# Autodesk Inventor assembly: Assembly1
(part 3 of 8)
- [Mate]: disk holder:43 ↔ Coil:85
- [Mate]: disk holder:43 ↔ Coil:85
- [Angle] (270 deg): disk holder:43 ↔ Coil:85
- [Mate]: disk holder:43 ↔ Coil:86
- [Angle] (270 deg): disk holder:43 ↔ Coil:86
- [Mate]: disk holder:43 ↔ Coil:86
- [RevoluteJoint]: disk holder:44 ↔ coin:44
- [Angle] (-25 deg): disk holder:44 ↔ coin:44
- [Mate]: disk holder:44 ↔ Coil:87
- [Mate]: disk holder:44 ↔ Coil:87
- [Angle] (270 deg): disk holder:44 ↔ Coil:87
- [Mate]: disk holder:44 ↔ Coil:88
- [Angle] (270 deg): disk holder:44 ↔ Coil:88
- [Mate]: disk holder:44 ↔ Coil:88
- [RevoluteJoint]: disk holder:45 ↔ coin:45
- [Angle] (-25 deg): disk holder:45 ↔ coin:45
- [Mate]: disk holder:45 ↔ Coil:89
- [Mate]: disk holder:45 ↔ Coil:89
- [Angle] (270 deg): disk holder:45 ↔ Coil:89
- [Mate]: disk holder:45 ↔ Coil:90
- [Angle] (270 deg): disk holder:45 ↔ Coil:90
- [Mate]: disk holder:45 ↔ Coil:90
- Flush:37: FRAME:1 ↔ disk holder:42
- Flush:38: FRAME:1 ↔ disk holder:43
- Flush:39: FRAME:1 ↔ disk holder:41
- Flush:40: FRAME:1 ↔ disk holder:38
- Mate:271: FRAME:1 ↔ disk holder:38
- Mate:272: FRAME:1 ↔ disk holder:38
- Flush:41: FRAME:1 ↔ disk holder:39
- Flush:42: FRAME:1 ↔ disk holder:45
- Flush:43: FRAME:1 ↔ disk holder:44
- Mate:277: FRAME:1 ↔ disk holder:44
- Mate:278: FRAME:1 ↔ disk holder:44
- Flush:44: FRAME:1 ↔ disk holder:40
- [RevoluteJoint]: disk holder:46 ↔ coin:46
- [Angle] (-25 deg): disk holder:46 ↔ coin:46
- [Mate]: disk holder:46 ↔ Coil:91
- [Mate]: disk holder:46 ↔ Coil:91
- [Angle] (270 deg): disk holder:46 ↔ Coil:91
- [Mate]: disk holder:46 ↔ Coil:92
- [Angle] (270 deg): disk holder:46 ↔ Coil:92
- [Mate]: disk holder:46 ↔ Coil:92
- [RevoluteJoint]: disk holder:47 ↔ coin:47
- [Angle] (-25 deg): disk holder:47 ↔ coin:47
- [Mate]: disk holder:47 ↔ Coil:93
- [Mate]: disk holder:47 ↔ Coil:93
- [Angle] (270 deg): disk holder:47 ↔ Coil:93
- [Mate]: disk holder:47 ↔ Coil:94
- [Angle] (270 deg): disk holder:47 ↔ Coil:94
- [Mate]: disk holder:47 ↔ Coil:94
- [RevoluteJoint]: disk holder:48 ↔ coin:48
- [Angle] (-25 deg): disk holder:48 ↔ coin:48
- [Mate]: disk holder:48 ↔ Coil:95
- [Mate]: disk holder:48 ↔ Coil:95
- [Angle] (270 deg): disk holder:48 ↔ Coil:95
- [Mate]: disk holder:48 ↔ Coil:96
- [Angle] (270 deg): disk holder:48 ↔ Coil:96
- [Mate]: disk holder:48 ↔ Coil:96
- [RevoluteJoint]: disk holder:50 ↔ coin:50
- [Angle] (-25 deg): disk holder:50 ↔ coin:50
- [Mate]: disk holder:50 ↔ Coil:99
- [Mate]: disk holder:50 ↔ Coil:99
- [Angle] (270 deg): disk holder:50 ↔ Coil:99
- [Mate]: disk holder:50 ↔ Coil:100
- [Angle] (270 deg): disk holder:50 ↔ Coil:100
- [Mate]: disk holder:50 ↔ Coil:100
- [RevoluteJoint]: disk holder:51 ↔ coin:51
- [Angle] (-25 deg): disk holder:51 ↔ coin:51
- [Mate]: disk holder:51 ↔ Coil:101
- [Mate]: disk holder:51 ↔ Coil:101
- [Angle] (270 deg): disk holder:51 ↔ Coil:101
- [Mate]: disk holder:51 ↔ Coil:102
- [Angle] (270 deg): disk holder:51 ↔ Coil:102
- [Mate]: disk holder:51 ↔ Coil:102
- [RevoluteJoint]: disk holder:53 ↔ coin:53
- [Angle] (-25 deg): disk holder:53 ↔ coin:53
- [Mate]: disk holder:53 ↔ Coil:105
- [Mate]: disk holder:53 ↔ Coil:105
- [Angle] (270 deg): disk holder:53 ↔ Coil:105
- [Mate]: disk holder:53 ↔ Coil:106
- [Angle] (270 deg): disk holder:53 ↔ Coil:106
- [Mate]: disk holder:53 ↔ Coil:106
- [RevoluteJoint]: disk holder:55 ↔ coin:55
- [Angle] (-25 deg): disk holder:55 ↔ coin:55
- [Mate]: disk holder:55 ↔ Coil:109
- [Mate]: disk holder:55 ↔ Coil:109
- [Angle] (270 deg): disk holder:55 ↔ Coil:109
- [Mate]: disk holder:55 ↔ Coil:110
- [Angle] (270 deg): disk holder:55 ↔ Coil:110
- [Mate]: disk holder:55 ↔ Coil:110
- [RevoluteJoint]: disk holder:57 ↔ coin:57
- [Angle] (-25 deg): disk holder:57 ↔ coin:57
- [Mate]: disk holder:57 ↔ Coil:113
- [Mate]: disk holder:57 ↔ Coil:113
- [Angle] (270 deg): disk holder:57 ↔ Coil:113
- [Mate]: disk holder:57 ↔ Coil:114
- [Angle] (270 deg): disk holder:57 ↔ Coil:114
- [Mate]: disk holder:57 ↔ Coil:114
- Flush:45: disk holder:46 ↔ disk holder:48
- Flush:46: disk holder:47 ↔ disk holder:48
- Flush:49: disk holder:50 ↔ disk holder:51
- Flush:59: disk holder:55 ↔ disk holder:57
- Flush:60: disk holder:53 ↔ disk holder:57
- Flush:61: disk holder:51 ↔ disk holder:55
- Flush:62: disk holder:50 ↔ disk holder:55
- Mate:335: FRAME:1 ↔ disk holder:48
- Mate:338: FRAME:1 ↔ disk holder:47
- Mate:339: FRAME:1 ↔ disk holder:55
- Mate:340: FRAME:1 ↔ disk holder:51
- Mate:343: FRAME:1 ↔ disk holder:53
- Mate:344: FRAME:1 ↔ disk holder:57
- Mate:345: FRAME:1 ↔ disk holder:50
- [RevoluteJoint]: disk holder:59 ↔ coin:59
- [Angle] (-25 deg): disk holder:59 ↔ coin:59
- [Mate]: disk holder:59 ↔ Coil:117
- [Mate]: disk holder:59 ↔ Coil:117
- [Angle] (270 deg): disk holder:59 ↔ Coil:117
- [Mate]: disk holder:59 ↔ Coil:118
- [Angle] (270 deg): disk holder:59 ↔ Coil:118
- [Mate]: disk holder:59 ↔ Coil:118
- [RevoluteJoint]: disk holder:60 ↔ coin:60
- [Angle] (-25 deg): disk holder:60 ↔ coin:60
- [Mate]: disk holder:60 ↔ Coil:119
- [Mate]: disk holder:60 ↔ Coil:119
- [Angle] (270 deg): disk holder:60 ↔ Coil:119
- [Mate]: disk holder:60 ↔ Coil:120
- [Angle] (270 deg): disk holder:60 ↔ Coil:120
- [Mate]: disk holder:60 ↔ Coil:120
- [RevoluteJoint]: disk holder:61 ↔ coin:61
- [Angle] (-25 deg): disk holder:61 ↔ coin:61
- [Mate]: disk holder:61 ↔ Coil:121
- [Mate]: disk holder:61 ↔ Coil:121
- [Angle] (270 deg): disk holder:61 ↔ Coil:121
- [Mate]: disk holder:61 ↔ Coil:122
- [Angle] (270 deg): disk holder:61 ↔ Coil:122
- [Mate]: disk holder:61 ↔ Coil:122
- [RevoluteJoint]: disk holder:62 ↔ coin:62
- [Angle] (-25 deg): disk holder:62 ↔ coin:62
- [Mate]: disk holder:62 ↔ Coil:123
- [Mate]: disk holder:62 ↔ Coil:123
- [Angle] (270 deg): disk holder:62 ↔ Coil:123
- [Mate]: disk holder:62 ↔ Coil:124
- [Angle] (270 deg): disk holder:62 ↔ Coil:124
- [Mate]: disk holder:62 ↔ Coil:124
- [RevoluteJoint]: disk holder:63 ↔ coin:63
- [Angle] (-25 deg): disk holder:63 ↔ coin:63
- [Mate]: disk holder:63 ↔ Coil:125
- [Mate]: disk holder:63 ↔ Coil:125
- [Angle] (270 deg): disk holder:63 ↔ Coil:125
- [Mate]: disk holder:63 ↔ Coil:126
- [Angle] (270 deg): disk holder:63 ↔ Coil:126
- [Mate]: disk holder:63 ↔ Coil:126
- [RevoluteJoint]: disk holder:64 ↔ coin:64
- [Angle] (-25 deg): disk holder:64 ↔ coin:64
- [Mate]: disk holder:64 ↔ Coil:127
- [Mate]: disk holder:64 ↔ Coil:127
- [Angle] (270 deg): disk holder:64 ↔ Coil:127
- [Mate]: disk holder:64 ↔ Coil:128
- [Angle] (270 deg): disk holder:64 ↔ Coil:128
- [Mate]: disk holder:64 ↔ Coil:128
- [RevoluteJoint]: disk holder:65 ↔ coin:65
- [Angle] (-25 deg): disk holder:65 ↔ coin:65
- [Mate]: disk holder:65 ↔ Coil:129
- [Mate]: disk holder:65 ↔ Coil:129
- [Angle] (270 deg): disk holder:65 ↔ Coil:129
- [Mate]: disk holder:65 ↔ Coil:130
- [Angle] (270 deg): disk holder:65 ↔ Coil:130
- [Mate]: disk holder:65 ↔ Coil:130
- [RevoluteJoint]: disk holder:66 ↔ coin:66
- [Angle] (-25 deg): disk holder:66 ↔ coin:66
- [Mate]: disk holder:66 ↔ Coil:131
- [Mate]: disk holder:66 ↔ Coil:131
- [Angle] (270 deg): disk holder:66 ↔ Coil:131
- [Mate]: disk holder:66 ↔ Coil:132
- [Angle] (270 deg): disk holder:66 ↔ Coil:132
- [Mate]: disk holder:66 ↔ Coil:132
- [RevoluteJoint]: disk holder:67 ↔ coin:67
- [Angle] (-25 deg): disk holder:67 ↔ coin:67
- [Mate]: disk holder:67 ↔ Coil:133
- [Mate]: disk holder:67 ↔ Coil:133
- [Angle] (270 deg): disk holder:67 ↔ Coil:133
- [Mate]: disk holder:67 ↔ Coil:134
- [Angle] (270 deg): disk holder:67 ↔ Coil:134
- [Mate]: disk holder:67 ↔ Coil:134
- [RevoluteJoint]: disk holder:68 ↔ coin:68
- [Angle] (-25 deg): disk holder:68 ↔ coin:68
- [Mate]: disk holder:68 ↔ Coil:135
- [Mate]: disk holder:68 ↔ Coil:135
- [Angle] (270 deg): disk holder:68 ↔ Coil:135
- [Mate]: disk holder:68 ↔ Coil:136
- [Angle] (270 deg): disk holder:68 ↔ Coil:136
- [Mate]: disk holder:68 ↔ Coil:136
- [RevoluteJoint]: disk holder:69 ↔ coin:69
- [Angle] (-25 deg): disk holder:69 ↔ coin:69
- [Mate]: disk holder:69 ↔ Coil:137
- [Mate]: disk holder:69 ↔ Coil:137
- [Angle] (270 deg): disk holder:69 ↔ Coil:137
- [Mate]: disk holder:69 ↔ Coil:138
- [Angle] (270 deg): disk holder:69 ↔ Coil:138
- [Mate]: disk holder:69 ↔ Coil:138
- Flush:71: disk holder:46 ↔ disk holder:61
- Flush:72: disk holder:61 ↔ disk holder:64
- Flush:73: disk holder:59 ↔ disk holder:64
- Flush:74: disk holder:59 ↔ disk holder:60
- Flush:75: disk holder:60 ↔ disk holder:62
- Flush:76: disk holder:60 ↔ disk holder:68
- Flush:77: disk holder:60 ↔ disk holder:63
- Flush:78: disk holder:63 ↔ disk holder:66
- Flush:79: disk holder:62 ↔ disk holder:65
- Flush:80: disk holder:65 ↔ disk holder:67
- Flush:81: disk holder:67 ↔ disk holder:69
- Flush:82: disk holder:46 ↔ disk holder:61
- Flush:83: disk holder:46 ↔ disk holder:62
- Flush:84: disk holder:46 ↔ disk holder:60
- Flush:85: disk holder:61 ↔ disk holder:65
- Flush:86: disk holder:64 ↔ disk holder:66
- Flush:88: disk holder:63 ↔ disk holder:67
- Flush:89: disk holder:68 ↔ disk holder:69
- Flush:90: disk holder:64 ↔ disk holder:67
- Flush:91: disk holder:64 ↔ disk holder:69
- Flush:92: disk holder:60 ↔ disk holder:67
- Mate:390: FRAME:1 ↔ disk holder:69
- Mate:391: FRAME:1 ↔ disk holder:69
- Mate:392: FRAME:1 ↔ disk holder:68
- Mate:393: FRAME:1 ↔ disk holder:61
- Mate:394: FRAME:1 ↔ disk holder:46
- Mate:395: FRAME:1 ↔ disk holder:60
- Mate:396: FRAME:1 ↔ disk holder:65
- Mate:397: FRAME:1 ↔ disk holder:62
- Mate:398: FRAME:1 ↔ disk holder:67
- Mate:399: FRAME:1 ↔ disk holder:63
- Mate:400: FRAME:1 ↔ disk holder:64
- Mate:401: FRAME:1 ↔ disk holder:66
- [RevoluteJoint]: disk holder:70 ↔ coin:70
- [Angle] (-25 deg): disk holder:70 ↔ coin:70
- [Mate]: disk holder:70 ↔ Coil:139
- [Mate]: disk holder:70 ↔ Coil:139
- [Angle] (270 deg): disk holder:70 ↔ Coil:139
- [Mate]: disk holder:70 ↔ Coil:140
- [Angle] (270 deg): disk holder:70 ↔ Coil:140
- [Mate]: disk holder:70 ↔ Coil:140
- [RevoluteJoint]: disk holder:71 ↔ coin:71
- [Angle] (-25 deg): disk holder:71 ↔ coin:71
- [Mate]: disk holder:71 ↔ Coil:141
- [Mate]: disk holder:71 ↔ Coil:141
- [Angle] (270 deg): disk holder:71 ↔ Coil:141
- [Mate]: disk holder:71 ↔ Coil:142
- [Angle] (270 deg): disk holder:71 ↔ Coil:142
- [Mate]: disk holder:71 ↔ Coil:142
- [RevoluteJoint]: disk holder:72 ↔ coin:72
- [Angle] (-25 deg): disk holder:72 ↔ coin:72
- [Mate]: disk holder:72 ↔ Coil:143
- [Mate]: disk holder:72 ↔ Coil:143
- [Angle] (270 deg): disk holder:72 ↔ Coil:143
- [Mate]: disk holder:72 ↔ Coil:144
- [Angle] (270 deg): disk holder:72 ↔ Coil:144
- [Mate]: disk holder:72 ↔ Coil:144
- [RevoluteJoint]: disk holder:74 ↔ coin:74
- [Angle] (-25 deg): disk holder:74 ↔ coin:74
- [Mate]: disk holder:74 ↔ Coil:147
- [Mate]: disk holder:74 ↔ Coil:147
- [Angle] (270 deg): disk holder:74 ↔ Coil:147
- [Mate]: disk holder:74 ↔ Coil:148
- [Angle] (270 deg): disk holder:74 ↔ Coil:148
- [Mate]: disk holder:74 ↔ Coil:148
- [RevoluteJoint]: disk holder:75 ↔ coin:75
- [Angle] (-25 deg): disk holder:75 ↔ coin:75
- [Mate]: disk holder:75 ↔ Coil:149
- [Mate]: disk holder:75 ↔ Coil:149
- [Angle] (270 deg): disk holder:75 ↔ Coil:149
- [Mate]: disk holder:75 ↔ Coil:150
- [Angle] (270 deg): disk holder:75 ↔ Coil:150
- [Mate]: disk holder:75 ↔ Coil:150
- [RevoluteJoint]: disk holder:76 ↔ coin:76
- [Angle] (-25 deg): disk holder:76 ↔ coin:76
- [Mate]: disk holder:76 ↔ Coil:151
- [Mate]: disk holder:76 ↔ Coil:151
- [Angle] (270 deg): disk holder:76 ↔ Coil:151
- [Mate]: disk holder:76 ↔ Coil:152
- [Angle] (270 deg): disk holder:76 ↔ Coil:152
- [Mate]: disk holder:76 ↔ Coil:152
- [RevoluteJoint]: disk holder:77 ↔ coin:77
- [Angle] (-25 deg): disk holder:77 ↔ coin:77
- [Mate]: disk holder:77 ↔ Coil:153
- [Mate]: disk holder:77 ↔ Coil:153
- [Angle] (270 deg): disk holder:77 ↔ Coil:153
- [Mate]: disk holder:77 ↔ Coil:154
- [Angle] (270 deg): disk holder:77 ↔ Coil:154
- [Mate]: disk holder:77 ↔ Coil:154
- [RevoluteJoint]: disk holder:78 ↔ coin:78
- [Angle] (-25 deg): disk holder:78 ↔ coin:78
- [Mate]: disk holder:78 ↔ Coil:155
- [Mate]: disk holder:78 ↔ Coil:155
- [Angle] (270 deg): disk holder:78 ↔ Coil:155
- [Mate]: disk holder:78 ↔ Coil:156
- [Angle] (270 deg): disk holder:78 ↔ Coil:156
- [Mate]: disk holder:78 ↔ Coil:156
- [RevoluteJoint]: disk holder:79 ↔ coin:79
- [Angle] (-25 deg): disk holder:79 ↔ coin:79
- [Mate]: disk holder:79 ↔ Coil:157
- [Mate]: disk holder:79 ↔ Coil:157
- [Angle] (270 deg): disk holder:79 ↔ Coil:157
- [Mate]: disk holder:79 ↔ Coil:158
- [Angle] (270 deg): disk holder:79 ↔ Coil:158
- [Mate]: disk holder:79 ↔ Coil:158
- [RevoluteJoint]: disk holder:80 ↔ coin:80
- [Angle] (-25 deg): disk holder:80 ↔ coin:80
- [Mate]: disk holder:80 ↔ Coil:159
- [Mate]: disk holder:80 ↔ Coil:159
- [Angle] (270 deg): disk holder:80 ↔ Coil:159
- [Mate]: disk holder:80 ↔ Coil:160
- [Angle] (270 deg): disk holder:80 ↔ Coil:160
- [Mate]: disk holder:80 ↔ Coil:160
- [RevoluteJoint]: disk holder:81 ↔ coin:81
- [Angle] (-25 deg): disk holder:81 ↔ coin:81
- [Mate]: disk holder:81 ↔ Coil:161
- [Mate]: disk holder:81 ↔ Coil:161
- [Angle] (270 deg): disk holder:81 ↔ Coil:161
- [Mate]: disk holder:81 ↔ Coil:162
- [Angle] (270 deg): disk holder:81 ↔ Coil:162
- [Mate]: disk holder:81 ↔ Coil:162
- Flush:94: disk holder:59 ↔ disk holder:74
- Flush:95: disk holder:74 ↔ disk holder:75
- Flush:96: disk holder:72 ↔ disk holder:74
- Flush:97: disk holder:59 ↔ disk holder:70
- Flush:98: disk holder:71 ↔ disk holder:74
- Flush:99: disk holder:72 ↔ disk holder:77
- Flush:100: disk holder:76 ↔ disk holder:77
- Flush:101: disk holder:77 ↔ disk holder:78
- Flush:102: disk holder:76 ↔ disk holder:79
- Flush:103: disk holder:80 ↔ disk holder:81
- Flush:104: disk holder:76 ↔ disk holder:80
- Flush:105: disk holder:78 ↔ disk holder:79
- Flush:106: disk holder:79 ↔ disk holder:81
- Flush:107: disk holder:77 ↔ disk holder:81
- Flush:108: disk holder:77 ↔ disk holder:80
- Flush:109: disk holder:76 ↔ disk holder:80
- Flush:110: disk holder:71 ↔ disk holder:76
- Flush:111: disk holder:71 ↔ disk holder:75
- Flush:112: disk holder:74 ↔ disk holder:75
- Flush:113: disk holder:72 ↔ disk holder:74
- Flush:114: disk holder:59 ↔ disk holder:72
- Mate:450: FRAME:1 ↔ disk holder:70
- Mate:451: FRAME:1 ↔ disk holder:74
- Mate:452: FRAME:1 ↔ disk holder:78
- Mate:453: FRAME:1 ↔ disk holder:77
- Mate:454: FRAME:1 ↔ disk holder:70
- Mate:455: FRAME:1 ↔ disk holder:72
- Mate:456: FRAME:1 ↔ disk holder:80
- Mate:457: FRAME:1 ↔ disk holder:81
- Mate:458: FRAME:1 ↔ disk holder:79
- Mate:459: FRAME:1 ↔ disk holder:75
- Mate:460: FRAME:1 ↔ disk holder:59
- Mate:461: FRAME:1 ↔ disk holder:71
- Mate:462: FRAME:1 ↔ disk holder:76
- [RevoluteJoint]: disk holder:82 ↔ coin:82
- [Angle] (-25 deg): disk holder:82 ↔ coin:82
- [Mate]: disk holder:82 ↔ Coil:163
- [Mate]: disk holder:82 ↔ Coil:163
- [Angle] (270 deg): disk holder:82 ↔ Coil:163
- [Mate]: disk holder:82 ↔ Coil:164
- [Angle] (270 deg): disk holder:82 ↔ Coil:164
- [Mate]: disk holder:82 ↔ Coil:164
- [RevoluteJoint]: disk holder:83 ↔ coin:83
- [Angle] (-25 deg): disk holder:83 ↔ coin:83
- [Mate]: disk holder:83 ↔ Coil:165
- [Mate]: disk holder:83 ↔ Coil:165
- [Angle] (270 deg): disk holder:83 ↔ Coil:165
- [Mate]: disk holder:83 ↔ Coil:166
- [Angle] (270 deg): disk holder:83 ↔ Coil:166
- [Mate]: disk holder:83 ↔ Coil:166
- [RevoluteJoint]: disk holder:84 ↔ coin:84
- [Angle] (-25 deg): disk holder:84 ↔ coin:84
- [Mate]: disk holder:84 ↔ Coil:167
- [Mate]: disk holder:84 ↔ Coil:167
- [Angle] (270 deg): disk holder:84 ↔ Coil:167
- [Mate]: disk holder:84 ↔ Coil:168
- [Angle] (270 deg): disk holder:84 ↔ Coil:168
- [Mate]: disk holder:84 ↔ Coil:168
- [RevoluteJoint]: disk holder:85 ↔ coin:85
- [Angle] (-25 deg): disk holder:85 ↔ coin:85
- [Mate]: disk holder:85 ↔ Coil:169
- [Mate]: disk holder:85 ↔ Coil:169
- [Angle] (270 deg): disk holder:85 ↔ Coil:169
- [Mate]: disk holder:85 ↔ Coil:170
- [Angle] (270 deg): disk holder:85 ↔ Coil:170
- [Mate]: disk holder:85 ↔ Coil:170
- [RevoluteJoint]: disk holder:86 ↔ coin:86
- [Angle] (-25 deg): disk holder:86 ↔ coin:86
- [Mate]: disk holder:86 ↔ Coil:171
- [Mate]: disk holder:86 ↔ Coil:171
- [Angle] (270 deg): disk holder:86 ↔ Coil:171
- [Mate]: disk holder:86 ↔ Coil:172
- [Angle] (270 deg): disk holder:86 ↔ Coil:172
- [Mate]: disk holder:86 ↔ Coil:172
- [RevoluteJoint]: disk holder:87 ↔ coin:87
- [Angle] (-25 deg): disk holder:87 ↔ coin:87
- [Mate]: disk holder:87 ↔ Coil:173
- [Mate]: disk holder:87 ↔ Coil:173
- [Angle] (270 deg): disk holder:87 ↔ Coil:173
- [Mate]: disk holder:87 ↔ Coil:174
- [Angle] (270 deg): disk holder:87 ↔ Coil:174
- [Mate]: disk holder:87 ↔ Coil:174
- [RevoluteJoint]: disk holder:88 ↔ coin:88
- [Angle] (-25 deg): disk holder:88 ↔ coin:88
- [Mate]: disk holder:88 ↔ Coil:175
- [Mate]: disk holder:88 ↔ Coil:175
- [Angle] (270 deg): disk holder:88 ↔ Coil:175
- [Mate]: disk holder:88 ↔ Coil:176
- [Angle] (270 deg): disk holder:88 ↔ Coil:176
- [Mate]: disk holder:88 ↔ Coil:176
- [RevoluteJoint]: disk holder:89 ↔ coin:89
- [Angle] (-25 deg): disk holder:89 ↔ coin:89
- [Mate]: disk holder:89 ↔ Coil:177
- [Mate]: disk holder:89 ↔ Coil:177
- [Angle] (270 deg): disk holder:89 ↔ Coil:177
- [Mate]: disk holder:89 ↔ Coil:178
- [Angle] (270 deg): disk holder:89 ↔ Coil:178
- [Mate]: disk holder:89 ↔ Coil:178
- [RevoluteJoint]: disk holder:90 ↔ coin:90
- [Angle] (-25 deg): disk holder:90 ↔ coin:90
- [Mate]: disk holder:90 ↔ Coil:179
- [Mate]: disk holder:90 ↔ Coil:179
- [Angle] (270 deg): disk holder:90 ↔ Coil:179
- [Mate]: disk holder:90 ↔ Coil:180
- [Angle] (270 deg): disk holder:90 ↔ Coil:180
- [Mate]: disk holder:90 ↔ Coil:180
- Flush:117: FRAME:1 ↔ disk holder:82
- Flush:118: disk holder:82 ↔ disk holder:83
- Flush:119: disk holder:83 ↔ disk holder:84
- Flush:120: disk holder:84 ↔ disk holder:85
- Flush:121: disk holder:85 ↔ disk holder:86
- Flush:122: disk holder:86 ↔ disk holder:87
- Flush:123: disk holder:87 ↔ disk holder:88
- Flush:124: disk holder:88 ↔ disk holder:89
- Flush:125: disk holder:89 ↔ disk holder:90
- Flush:126: disk holder:82 ↔ disk holder:83
- Flush:127: disk holder:83 ↔ disk holder:84
- Flush:128: disk holder:84 ↔ disk holder:85
- Flush:129: disk holder:85 ↔ disk holder:86
- Flush:130: disk holder:86 ↔ disk holder:87
- Flush:131: disk holder:87 ↔ disk holder:88
- Flush:132: disk holder:88 ↔ disk holder:89
- Flush:133: disk holder:89 ↔ disk holder:90
- Mate:499: FRAME:1 ↔ disk holder:82
- Mate:500: FRAME:1 ↔ disk holder:82
- Mate:501: FRAME:1 ↔ disk holder:83
- Mate:502: FRAME:1 ↔ disk holder:84
- Mate:503: FRAME:1 ↔ disk holder:85
- Mate:504: FRAME:1 ↔ disk holder:86
- Mate:505: FRAME:1 ↔ disk holder:87
- Mate:506: FRAME:1 ↔ disk holder:88
- Mate:507: FRAME:1 ↔ disk holder:89
- Mate:508: FRAME:1 ↔ disk holder:90
- [RevoluteJoint]: disk holder:91 ↔ coin:91
- [Angle] (-25 deg): disk holder:91 ↔ coin:91
- [Mate]: disk holder:91 ↔ Coil:181
- [Mate]: disk holder:91 ↔ Coil:181
- [Angle] (270 deg): disk holder:91 ↔ Coil:181
- [Mate]: disk holder:91 ↔ Coil:182
- [Angle] (270 deg): disk holder:91 ↔ Coil:182
- [Mate]: disk holder:91 ↔ Coil:182
- Flush:134: FRAME:1 ↔ disk holder:91
- Mate:513: FRAME:1 ↔ disk holder:91
- Mate:514: FRAME:1 ↔ disk holder:91
- [RevoluteJoint]: disk holder:92 ↔ coin:92
- [Angle] (-25 deg): disk holder:92 ↔ coin:92
- [Mate]: disk holder:92 ↔ Coil:183
- [Mate]: disk holder:92 ↔ Coil:183
- [Angle] (270 deg): disk holder:92 ↔ Coil:183
- [Mate]: disk holder:92 ↔ Coil:184
- [Angle] (270 deg): disk holder:92 ↔ Coil:184
- [Mate]: disk holder:92 ↔ Coil:184
- [RevoluteJoint]: disk holder:93 ↔ coin:93
- [Angle] (-25 deg): disk holder:93 ↔ coin:93
- [Mate]: disk holder:93 ↔ Coil:185
- [Mate]: disk holder:93 ↔ Coil:185
- [Angle] (270 deg): disk holder:93 ↔ Coil:185
- [Mate]: disk holder:93 ↔ Coil:186
- [Angle] (270 deg): disk holder:93 ↔ Coil:186
- [Mate]: disk holder:93 ↔ Coil:186
- [RevoluteJoint]: disk holder:94 ↔ coin:94
- [Angle] (-25 deg): disk holder:94 ↔ coin:94
- [Mate]: disk holder:94 ↔ Coil:187
- [Mate]: disk holder:94 ↔ Coil:187
- [Angle] (270 deg): disk holder:94 ↔ Coil:187